# Autodesk Inventor assembly: Swarmie
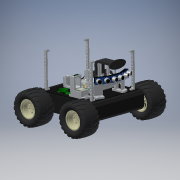
[picture p0: Inventor's stored thumbnail of the model, 180x180]
Saved by Autodesk Inventor 2016 (Build 200138000, 138)
## iProperties
Created: 2015-08-28
Part Number: Swarmie
Document SubType Name: Assembly
Designer: lachesis
Author: lachesis
## Documents named in this file (15)
- C:\Users\lachesis\git\Swarmie-Build\Swarmie-Assembly\Assemblies\Swarmie.iam
- C:\Users\lachesis\git\Swarmie-Build\Swarmie-Assembly\Assemblies\Chassis.iam
- C:\Users\lachesis\git\Swarmie-Build\Swarmie-Assembly\Parts\DCMotor.ipt
- C:\Users\lachesis\git\Swarmie-Build\Swarmie-Assembly\Parts\MotorHub.ipt
- C:\Users\lachesis\git\Swarmie-Build\Swarmie-Assembly\Parts\TireWheelRight.ipt
- C:\Users\lachesis\git\Swarmie-Build\Swarmie-Assembly\Parts\CoverPlate.ipt
- C:\Users\lachesis\git\Swarmie-Build\Swarmie-Assembly\Assemblies\TopPlate.iam
- C:\Users\lachesis\git\Swarmie-Build\Swarmie-Assembly\Parts\LidSupportLW.ipt
- C:\Users\lachesis\git\Swarmie-Build\Swarmie-Assembly\Parts\NUC.ipt
- C:\Users\lachesis\git\Swarmie-Build\Swarmie-Assembly\Parts\Ultrasound.ipt
- C:\Users\lachesis\git\Swarmie-Build\Swarmie-Assembly\Parts\Camera.ipt
- C:\Users\lachesis\git\Swarmie-Build\Swarmie-Assembly\Parts\TireWheelLeft.ipt
- C:\Users\lachesis\git\Swarmie-Build\Swarmie-Assembly\Parts\IMU.ipt
- C:\Users\lachesis\git\Swarmie-Build\Swarmie-Assembly\Parts\GPS.ipt
- C:\Users\lachesis\git\Swarmie-Build\Swarmie-Assembly\Assemblies\BottomPlate.iam
## Components (27 placed, 14 different names)
1. Chassis:1 [sub-assembly] — Rigid:4, Rigid:20, Rigid:18, Rigid:15, Rigid:9, Rigid:33
2. DCMotor:1 — Rigid:15, Rigid:16
3. DCMotor:2 — Rigid:4, Rigid:17
4. DCMotor:3 — Rigid:18, Rigid:19
5. DCMotor:4 — Rigid:20, Rigid:21
6. MotorHub:1 — Rigid:16, Rigid:30
7. MotorHub:2 — Rigid:19, Rigid:31
8. MotorHub:3 — Rigid:21, Rigid:8
9. MotorHub:4 — Rigid:17, Rigid:7
10. TireWheelLeft:1 — Rigid:31
11. TireWheelLeft:2 — Rigid:30
12. TireWheelRight:3 — Rigid:7
13. TireWheelRight:4 — Rigid:8
14. TopPlate:1 [sub-assembly] — Rigid:9, Rigid:10, Rigid:12, Rigid:13, Rigid:23, Rigid:25, Rigid:26, Rigid:27, Rigid:28, Mate:1, Mate:2, Rigid:32, Mate:3, Flush:1, Mate:4
15. LidSupportLW:1 — Rigid:13
16. LidSupportLW:2 — Rigid:12
17. LidSupportLW:3 — Rigid:23
18. LidSupportLW:4 — Rigid:10, Rigid:24
19. CoverPlate:1 — Rigid:24
20. NUC:1 — Rigid:25
21. Ultrasound:1 — Rigid:26
22. Ultrasound:2 — Rigid:27
23. Ultrasound:3 — Rigid:28
24. Camera:1 — Mate:1, Mate:2
25. IMU:1 — Rigid:32
26. GPS:1 — Mate:3, Flush:1, Mate:4
27. BottomPlate:1 [sub-assembly] — Rigid:33
## Relationships (29: WeldJoint 24, Mate 4, Flush 1)
- Rigid:4 [WeldJoint]: Chassis:1 ↔ DCMotor:2
- Rigid:20 [WeldJoint]: Chassis:1 ↔ DCMotor:4
- Rigid:18 [WeldJoint]: Chassis:1 ↔ DCMotor:3
- Rigid:15 [WeldJoint]: Chassis:1 ↔ DCMotor:1
- Rigid:16 [WeldJoint] (2.54 mm): DCMotor:1 ↔ MotorHub:1
- Rigid:19 [WeldJoint] (2.54 mm): DCMotor:3 ↔ MotorHub:2
- Rigid:21 [WeldJoint] (2.54 mm): DCMotor:4 ↔ MotorHub:3
- Rigid:17 [WeldJoint] (-2.54 mm): DCMotor:2 ↔ MotorHub:4
- Rigid:7 [WeldJoint]: MotorHub:4 ↔ TireWheelRight:3
- Rigid:8 [WeldJoint]: MotorHub:3 ↔ TireWheelRight:4
- Rigid:9 [WeldJoint]: Chassis:1 ↔ TopPlate:1
- Rigid:10 [WeldJoint]: TopPlate:1 ↔ LidSupportLW:4
- Rigid:12 [WeldJoint]: TopPlate:1 ↔ LidSupportLW:2
- Rigid:13 [WeldJoint]: TopPlate:1 ↔ LidSupportLW:1
- Rigid:23 [WeldJoint]: TopPlate:1 ↔ LidSupportLW:3
- Rigid:24 [WeldJoint]: LidSupportLW:4 ↔ CoverPlate:1
- Rigid:25 [WeldJoint]: TopPlate:1 ↔ NUC:1
- Rigid:26 [WeldJoint]: TopPlate:1 ↔ Ultrasound:1
- Rigid:27 [WeldJoint]: TopPlate:1 ↔ Ultrasound:2
- Rigid:28 [WeldJoint]: TopPlate:1 ↔ Ultrasound:3
- Mate:1: TopPlate:1 ↔ Camera:1
- Mate:2: TopPlate:1 ↔ Camera:1
- Rigid:30 [WeldJoint]: MotorHub:1 ↔ TireWheelLeft:2
- Rigid:31 [WeldJoint]: MotorHub:2 ↔ TireWheelLeft:1
- Rigid:32 [WeldJoint]: TopPlate:1 ↔ IMU:1
- Mate:3: TopPlate:1 ↔ GPS:1
- Flush:1: TopPlate:1 ↔ GPS:1
- Mate:4: TopPlate:1 ↔ GPS:1
- Rigid:33 [WeldJoint]: Chassis:1 ↔ BottomPlate:1
